# Autodesk Inventor assembly: Robot
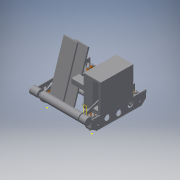
[picture p0: Inventor's stored thumbnail of the model, 180x180]
Saved by Autodesk Inventor 2017 (Build 210142000, 142)
## iProperties
Created: 2016-10-08
Part Number: Robot
Document SubType Name: Assembly
Designer: RoboticsUser
Author: RoboticsUser
## Documents named in this file (7)
- C:\Robotics\CAD\2016-17_CAD\Robot - CAD.iam
- C:\Robotics\CAD\COTSParts\Bosch Extrusion\Bosch 20x20 9 in - Copy.ipt
- C:\Robotics\CAD\2016-17_CAD\WheelAssemble2.0.iam
- C:\Robotics\CAD\COTSParts\Bosch Extrusion\Bosch 20x20 9 real.ipt
- C:\Robotics\CAD\2016-17_CAD\CollectorHolderAssembly.iam
- C:\Robotics\CAD\2016-17_CAD\UpProto.ipt
- C:\Robotics\CAD\2016-17_CAD\ShooterProto.ipt
## Components (10 placed, 6 different names)
1. Bosch 20x20 9 in - Copy:1 — Flush:150, Mate:248, Flush:151, Flush:152, Mate:251, Flush:156, Flush:157, Mate:252, Flush:158, Mate:254, Flush:161
2. Bosch 20x20 9 in - Copy:2 — Mate:249, Flush:153, Flush:154, Mate:250, Flush:155, Flush:159, Mate:253, Flush:160
3. WheelAssemble2.0:1 [sub-assembly] — Flush:154, Mate:250, Flush:155, Mate:253, Flush:160, Flush:162, Mate:256, Flush:166, Flush:167, Mate:261, Mate:262, Flush:169, Flush:170, Mate:263, Mate:265, Mate:266
4. WheelAssemble2.0:2 [sub-assembly] — Flush:150, Mate:252, Flush:158, Mate:254, Flush:161, Flush:163
5. Bosch 20x20 9 real:1 — Mate:251, Flush:156, Flush:157, Mate:257
6. Bosch 20x20 9 real:2 — Mate:248, Flush:151, Flush:152, Mate:249, Flush:153, Flush:159, Flush:162, Flush:163
7. CollectorHolderAssembly:1 [sub-assembly] — Mate:256, Flush:166, Flush:167
8. UpProto:1 — Mate:261, Mate:263, Mate:264, Mate:265, Mate:266, Flush:171, Mate:267
9. UpProto:2 — Mate:257, Flush:171, Mate:267
10. ShooterProto:1 — Mate:262, Flush:169, Flush:170, Mate:264
## Relationships (35: Flush 19, Mate 16)
- Flush:150: Bosch 20x20 9 in - Copy:1 ↔ WheelAssemble2.0:2
- Mate:248: Bosch 20x20 9 in - Copy:1 ↔ Bosch 20x20 9 real:2
- Flush:151: Bosch 20x20 9 in - Copy:1 ↔ Bosch 20x20 9 real:2
- Flush:152: Bosch 20x20 9 in - Copy:1 ↔ Bosch 20x20 9 real:2
- Mate:249: Bosch 20x20 9 in - Copy:2 ↔ Bosch 20x20 9 real:2
- Flush:153: Bosch 20x20 9 in - Copy:2 ↔ Bosch 20x20 9 real:2
- Flush:154: Bosch 20x20 9 in - Copy:2 ↔ WheelAssemble2.0:1
- Mate:250: Bosch 20x20 9 in - Copy:2 ↔ WheelAssemble2.0:1
- Flush:155 (-38.1 mm): Bosch 20x20 9 in - Copy:2 ↔ WheelAssemble2.0:1
- Mate:251: Bosch 20x20 9 in - Copy:1 ↔ Bosch 20x20 9 real:1
- Flush:156: Bosch 20x20 9 in - Copy:1 ↔ Bosch 20x20 9 real:1
- Flush:157: Bosch 20x20 9 in - Copy:1 ↔ Bosch 20x20 9 real:1
- Mate:252: Bosch 20x20 9 in - Copy:1 ↔ WheelAssemble2.0:2
- Flush:158 (38.1 mm): Bosch 20x20 9 in - Copy:1 ↔ WheelAssemble2.0:2
- Flush:159: Bosch 20x20 9 in - Copy:2 ↔ Bosch 20x20 9 real:2
- Mate:253: Bosch 20x20 9 in - Copy:2 ↔ WheelAssemble2.0:1
- Mate:254: Bosch 20x20 9 in - Copy:1 ↔ WheelAssemble2.0:2
- Flush:160: Bosch 20x20 9 in - Copy:2 ↔ WheelAssemble2.0:1
- Flush:161: Bosch 20x20 9 in - Copy:1 ↔ WheelAssemble2.0:2
- Flush:162 (38.1 mm): WheelAssemble2.0:1 ↔ Bosch 20x20 9 real:2
- Flush:163 (38.1 mm): WheelAssemble2.0:2 ↔ Bosch 20x20 9 real:2
- Mate:256: WheelAssemble2.0:1 ↔ CollectorHolderAssembly:1
- Flush:166 (128.905 mm): WheelAssemble2.0:1 ↔ CollectorHolderAssembly:1
- Flush:167: WheelAssemble2.0:1 ↔ CollectorHolderAssembly:1
- Mate:257: Bosch 20x20 9 real:1 ↔ UpProto:2
- Mate:261: WheelAssemble2.0:1 ↔ UpProto:1
- Mate:262: WheelAssemble2.0:1 ↔ ShooterProto:1
- Flush:169: WheelAssemble2.0:1 ↔ ShooterProto:1
- Flush:170 (69.85 mm): WheelAssemble2.0:1 ↔ ShooterProto:1
- Mate:263: WheelAssemble2.0:1 ↔ UpProto:1
- Mate:264: UpProto:1 ↔ ShooterProto:1
- Mate:265: WheelAssemble2.0:1 ↔ UpProto:1
- Mate:266 (370.84 mm): WheelAssemble2.0:1 ↔ UpProto:1
- Flush:171: UpProto:1 ↔ UpProto:2
- Mate:267 (95.25 mm): UpProto:1 ↔ UpProto:2
